# Autodesk Inventor assembly: Bumper
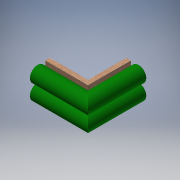
[picture p0: Inventor's stored thumbnail of the model, 180x180]
Saved by Autodesk Inventor 2017 (Build 210142000, 142)
## iProperties
Created: 2017-02-12
Part Number: Bumper
Document SubType Name: Assembly
Designer: kingb
Author: kingb
## Documents named in this file (4)
- C:\Users\kingb\Desktop\CAD\Bumper.iam
- C:\Users\kingb\Desktop\CAD\D1.ipt
- C:\Users\kingb\Desktop\CAD\D2.ipt
- C:\Users\kingb\Desktop\CAD\Pool Noodle.ipt
## Components (6 placed, 3 different names)
1. D1:1 — Mate:1, Flush:1, Mate:2, Tangent:2, Flush:3, Tangent:4
2. D2:1 — Mate:1, Flush:1, Mate:2, Tangent:1, Flush:2, Tangent:3, Tangent:7
3. Pool Noodle:3 — Tangent:1, Flush:2, Mate:3, Mate:4, Tangent:6, Tangent:7
4. Pool Noodle:4 — Mate:3, Tangent:2, Mate:4, Flush:3, Tangent:5
5. Pool Noodle:5 — Tangent:3, Tangent:6
6. Pool Noodle:6 — Tangent:4, Tangent:5
## Relationships (16: Tangent 7, Mate 6, Flush 3)
- Mate:1: D1:1 ↔ D2:1
- Flush:1: D1:1 ↔ D2:1
- Mate:2: D1:1 ↔ D2:1
- Tangent:1: D2:1 ↔ Pool Noodle:3
- Flush:2: D2:1 ↔ Pool Noodle:3
- Mate:3: Pool Noodle:3 ↔ Pool Noodle:4
- Tangent:2: D1:1 ↔ Pool Noodle:4
- Mate:4: Pool Noodle:3 ↔ Pool Noodle:4
- Flush:3: D1:1 ↔ Pool Noodle:4
- [Mate]: Pool Noodle:5 ↔ Pool Noodle:6
- [Mate]: Pool Noodle:5 ↔ Pool Noodle:6
- Tangent:3: D2:1 ↔ Pool Noodle:5
- Tangent:4: D1:1 ↔ Pool Noodle:6
- Tangent:5: Pool Noodle:4 ↔ Pool Noodle:6
- Tangent:6: Pool Noodle:3 ↔ Pool Noodle:5
- Tangent:7: D2:1 ↔ Pool Noodle:3
## Named parameters: d12_d8 = 0 mm, d13_d10 = 0 mm
